# Autodesk Inventor assembly: HbSocketU02
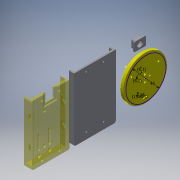
[picture p0: Inventor's stored thumbnail of the model, 180x180]
Saved by Autodesk Inventor 2016 (Build 200138000, 138)
## iProperties
Created: 2015-02-09
Part Number: HbSocketU02
Document SubType Name: Assembly
Designer: Yamaura
Author: Yamaura
## Documents named in this file (13)
- C:\Users\Yamaura\Documents\GitHub\HACKberry\HACKberry-hardware\3D\Inventor\HACKberry_v1_for_print7.iam
- C:\Users\Yamaura\Documents\GitHub\HACKberry\HACKberry-hardware\3D\Inventor\Parts\HbBatteryDoor03.ipt
- C:\Users\Yamaura\Documents\GitHub\HACKberry\HACKberry-hardware\3D\Inventor\Parts\HbBatteryDoorKnob03.ipt
- C:\Users\Yamaura\Documents\GitHub\HACKberry\HACKberry-hardware\3D\Inventor\Parts\HbBatteryHingeA03.ipt
- C:\Users\Yamaura\Documents\GitHub\HACKberry\HACKberry-hardware\3D\Inventor\Parts\HbBatteryHingeB03.ipt
- C:\Users\Yamaura\Documents\GitHub\HACKberry\HACKberry-hardware\3D\Inventor\Parts\HbBatteryHingeC03.ipt
- C:\Users\Yamaura\Documents\GitHub\HACKberry\HACKberry-hardware\3D\Inventor\Parts\HbBatteryCase01.ipt
- C:\Users\Yamaura\Documents\GitHub\HACKberry\HACKberry-hardware\3D\Inventor\Parts\HbBatteryLockKnob01.ipt
- C:\Users\Yamaura\Documents\GitHub\HACKberry\HACKberry-hardware\3D\Inventor\Parts\HbBatteryDoorLever03.ipt
- C:\Users\Yamaura\Documents\GitHub\HACKberry\HACKberry-hardware\3D\Inventor\Parts\HbMainFrameA01.ipt
- C:\Users\Yamaura\Documents\GitHub\HACKberry\HACKberry-hardware\3D\Inventor\Parts\HbMainFrameB01.ipt
- C:\Users\Yamaura\Documents\GitHub\HACKberry\HACKberry-hardware\3D\Inventor\Parts\HbBatteryCaseBottom01.ipt
- C:\Users\Yamaura\Documents\GitHub\HACKberry\HACKberry-hardware\3D\Inventor\Parts\HbWristLockPlate01.ipt
## Components (12 placed, 12 different names)
1. HbBatteryDoorKnob03:1
2. HbBatteryCase01:1 — フラッシュ:1, フラッシュ:2, メイト:1, フラッシュ:3, フラッシュ:4
3. HbBatteryLockKnob01:1 — フラッシュ:4
4. HbBatteryHingeC03:1
5. HbBatteryHingeB03:1
6. HbBatteryHingeA03:1
7. HbBatteryDoor03:1
8. HbMainFrameA01:1
9. HbMainFrameB01:1
10. HbBatteryDoorLever03:1
11. HbBatteryCaseBottom01:1 — フラッシュ:1, フラッシュ:2, メイト:1
12. HbWristLockPlate01:1 — フラッシュ:3
## Relationships (5: Flush 4, Mate 1)
- フラッシュ:1 [Flush]: HbBatteryCase01:1 ↔ HbBatteryCaseBottom01:1
- フラッシュ:2 [Flush]: HbBatteryCase01:1 ↔ HbBatteryCaseBottom01:1
- メイト:1 [Mate] (5 mm): HbBatteryCase01:1 ↔ HbBatteryCaseBottom01:1
- フラッシュ:3 [Flush]: HbBatteryCase01:1 ↔ HbWristLockPlate01:1
- フラッシュ:4 [Flush]: HbBatteryCase01:1 ↔ HbBatteryLockKnob01:1
